# Autodesk Inventor assembly: Transducer
Saved by Autodesk Inventor 2021 (Build 250183000, 183)
## iProperties
Created: 2021-01-20
Part Number: Transducer
Document SubType Name: Assembly
Designer: User
Author: User
## Documents named in this file (3)
- D:\SynologyDrive\tcodev\tco-cad\common\hcsr04\Transducer.iam
- D:\SynologyDrive\tcodev\tco-cad\common\hcsr04\TransducerBody.ipt
- D:\SynologyDrive\tcodev\tco-cad\common\hcsr04\Mesh.ipt
## Components (2 placed, 2 different names)
1. TransducerBody:1 — Mate:1, Mate:2
2. Mesh:1 — Mate:1, Mate:2
## Relationships (2: Mate 2)
- Mate:1: TransducerBody:1 ↔ Mesh:1
- Mate:2: TransducerBody:1 ↔ Mesh:1
